# Autodesk Inventor assembly: RCUAssy
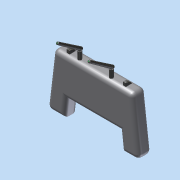
[picture p0: Inventor's stored thumbnail of the model, 180x180]
Saved by Autodesk Inventor 2011 SP1 (Build 150282100, 282)
## iProperties
Created: 2011-08-15
Part Number: RCUAssy
Document SubType Name: Assembly
Designer: dgitz
Author: dgitz
## Documents named in this file (4)
- C:\Dropbox\ICARUS\Remote Control Unit (RCU)\RCU v2\Design\RCUv2-3\RCUAssy.iam
- C:\Dropbox\ICARUS\Remote Control Unit (RCU)\RCU v2\Design\RCUv2-3\RUCBase.ipt
- C:\Dropbox\ICARUS\Remote Control Unit (RCU)\RCU v2\Design\Library\Trigger.ipt
- C:\Dropbox\ICARUS\Remote Control Unit (RCU)\RCU v2\Design\Library\XBeeAntennaAssy.iam
## Components (5 placed, 3 different names)
1. RUCBase:1 — Mate:1, Angle:1, Mate:4, Mate:5, Mate:6, Mate:7, Angle:2, Angle:3
2. Trigger:1 — Mate:1, Mate:2, Flush:1, Mate:3, Angle:1
3. Trigger:2 — Mate:2, Flush:1, Mate:3
4. XBeeAntennaAssy:1 [sub-assembly] — Mate:4, Mate:7, Angle:2
5. XBeeAntennaAssy:2 [sub-assembly] — Mate:5, Mate:6, Angle:3
## Relationships (11: Mate 7, Angle 3, Flush 1)
- Mate:1: RUCBase:1 ↔ Trigger:1
- Mate:2: Trigger:1 ↔ Trigger:2
- Flush:1: Trigger:1 ↔ Trigger:2
- Mate:3 (152.4 mm): Trigger:1 ↔ Trigger:2
- Angle:1 (270 deg): RUCBase:1 ↔ Trigger:1
- Mate:4: RUCBase:1 ↔ XBeeAntennaAssy:1
- Mate:5: RUCBase:1 ↔ XBeeAntennaAssy:2
- Mate:6 (-12.7 mm): RUCBase:1 ↔ XBeeAntennaAssy:2
- Mate:7 (-12.7 mm): RUCBase:1 ↔ XBeeAntennaAssy:1
- Angle:2 (145 deg): RUCBase:1 ↔ XBeeAntennaAssy:1
- Angle:3 (145 deg): RUCBase:1 ↔ XBeeAntennaAssy:2
